# Autodesk Inventor assembly: New Mixer Cover 2
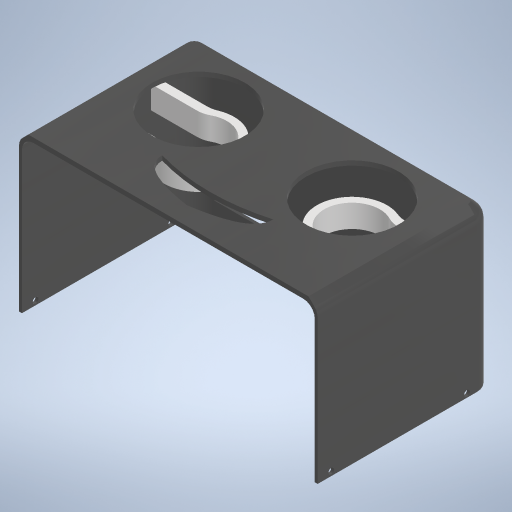
[picture p0: Inventor's stored thumbnail of the model, 512x512]
Saved by Autodesk Inventor 2024.3 (Build 283343010, 343A)
## iProperties
Created: 2025-04-07
Part Number: New Mixer Cover 2
Document SubType Name: Assembly
Designer: Vincent Larson
Author: Vincent Larson
## Documents named in this file (3)
- C:\Users\Vincent Larson\Downloads\Bubba ipt-iam files\Bubba Head\New Mixer Cover 2.iam
- C:\Users\Vincent Larson\Downloads\Bubba ipt-iam files\Bubba Head\Mixer and nozzle cover copy.ipt
- C:\Users\Vincent Larson\Downloads\Bubba ipt-iam files\Bubba Head\eye motor holder2.ipt
## Components (3 placed, 2 different names)
1. Mixer and nozzle cover copy:1 — Mate:1, Mate:2, Mate:3, Flush:1, Mate:4, Flush:2
2. eye motor holder2:1 — Mate:2, Mate:3, Flush:1
3. eye motor holder2:2 — Mate:1, Mate:4, Flush:2
## Relationships (6: Mate 4, Flush 2)
- Mate:1: Mixer and nozzle cover copy:1 ↔ eye motor holder2:2
- Mate:2: Mixer and nozzle cover copy:1 ↔ eye motor holder2:1
- Mate:3 (8.382 mm): Mixer and nozzle cover copy:1 ↔ eye motor holder2:1
- Flush:1 (33.274 mm): Mixer and nozzle cover copy:1 ↔ eye motor holder2:1
- Mate:4 (8.382 mm): Mixer and nozzle cover copy:1 ↔ eye motor holder2:2
- Flush:2 (33.274 mm): Mixer and nozzle cover copy:1 ↔ eye motor holder2:2
